# Autodesk Inventor assembly: B3M-SC-1170-A_with_ClampHorn_AND_FreeHorn
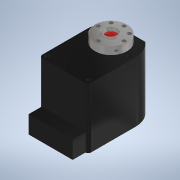
[picture p0: Inventor's stored thumbnail of the model, 180x180]
Saved by Autodesk Inventor 2020.4 (Build 244396000, 396)
## iProperties
Created: 2022-03-18
Part Number: B3M-SC-1170-A_with_ClampHorn_AND_FreeHorn
Document SubType Name: Assembly
Designer: MasatoKubotera
Author: MasatoKubotera
## Documents named in this file (5)
- C:\Users\Masato\Desktop\SUSTAINA-OP\ReadyMade\KONDO\B3M-SC-1170-A_with_ClampHorn_AND_FreeHorn.iam
- C:\Users\Masato\Desktop\SUSTAINA-OP\ReadyMade\KONDO\B3M-SC-1170-A_with_ClampHorn.iam
- C:\Users\Masato\Desktop\SUSTAINA-OP\ReadyMade\KONDO\FreeHorn.ipt
- C:\Users\Masato\Desktop\SUSTAINA-OP\ReadyMade\KONDO\FreeHorn_Screw.ipt
- C:\Users\Masato\Desktop\SUSTAINA-OP\ReadyMade\Washer\TT-1220-20.ipt
## Components (4 placed, 4 different names)
1. B3M-SC-1170-A_with_ClampHorn:1 [sub-assembly] — 挿入:1, 挿入:2, フラッシュ:1, フラッシュ:2, フラッシュ:4
2. FreeHorn_:1 — 挿入:1, 挿入:3
3. FreeHorn_Screw:1 — 挿入:2
4. TT-1220-20:1 — 挿入:3
## Relationships (7: Flush 4, Insert 3)
- 挿入:1 [Insert]: B3M-SC-1170-A_with_ClampHorn:1 ↔ FreeHorn_:1
- 挿入:2 [Insert]: B3M-SC-1170-A_with_ClampHorn:1 ↔ FreeHorn_Screw:1
- フラッシュ:1 [Flush]: B3M-SC-1170-A_with_ClampHorn:1
- フラッシュ:2 [Flush]: B3M-SC-1170-A_with_ClampHorn:1
- フラッシュ:3 [Flush]
- フラッシュ:4 [Flush] (-19.75 mm): B3M-SC-1170-A_with_ClampHorn:1
- 挿入:3 [Insert]: FreeHorn_:1 ↔ TT-1220-20:1
